# Autodesk Inventor assembly: Ствол
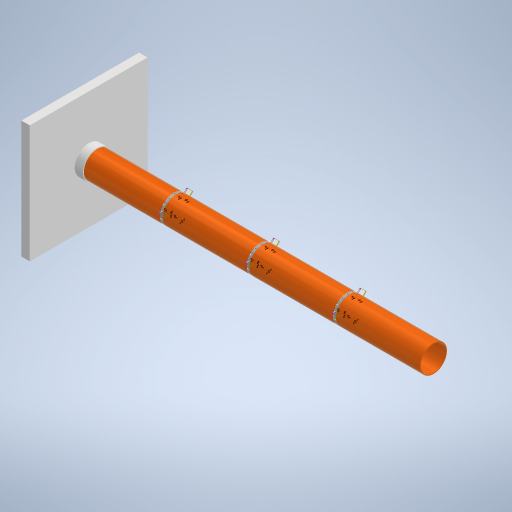
[picture p0: Inventor's stored thumbnail of the model, 512x512]
Saved by Autodesk Inventor 2023 (Build 270158000, 158)
## iProperties
Created: 2024-01-16
Part Number: Ствол
Document SubType Name: Assembly
Designer: liza
Author: liza
## Documents named in this file (6)
- C:\Fox_Crow\Work\Crow_Sborka\Ствол.iam
- C:\Fox_Crow\Work\Crow_Sborka\труба.ipt
- C:\Fox_Crow\Work\Crow_Sborka\внутренний соеденитель труб2.ipt
- C:\Fox_Crow\Work\Crow_Sborka\ветка.ipt
- C:\Fox_Crow\Work\Crow_Sborka\крепеж крышки+доска.ipt
- C:\Fox_Crow\Work\Crow_Sborka\трубка ветка.ipt
## Components (24 placed, 5 different names)
1. ветка:1 — Заподлицо:2
2. крепеж крышки+доска:1 — Цилиндрический:1, С поворотом:1
3. труба:5 — С поворотом:2
4. труба:2 — Совмещение:1, Совмещение:2, Заподлицо:1, Совмещение:3, Совмещение:4, Цилиндрический:1, С поворотом:1
5. труба:3
6. труба:4 — С поворотом:2
7. внутренний соеденитель труб2:1 — Совмещение:3, Совмещение:4, Цилиндрический:2, Цилиндрический:3
8. трубка ветка:1 — Цилиндрический:2, Цилиндрический:3
9. внутренний соеденитель труб2:2
10. трубка ветка:3
11. внутренний соеденитель труб2:3
12. трубка ветка:4
13. внутренний соеденитель труб2:4
14. трубка ветка:5
15. внутренний соеденитель труб2:5
16. трубка ветка:6
17. внутренний соеденитель труб2:6
18. трубка ветка:7
19. внутренний соеденитель труб2:7
20. трубка ветка:8
21. внутренний соеденитель труб2:8
22. трубка ветка:9
23. внутренний соеденитель труб2:9
24. трубка ветка:10
## Component patterns: (3 elements, first: труба:2), (1 elements), МассивКомп 2:2 (1 elements), МассивКомп 2:3 (1 elements), (3 elements, first: внутренний соеденитель труб2:1 + трубка ветка:1), МассивКомп 1:2 (3 elements), МассивКомп 1:3 (3 elements)
## Relationships (11: Mate 4, CylindricalJoint 3, Flush 2, RevoluteJoint 2)
- Совмещение:1 [Mate]: труба:2
- Совмещение:2 [Mate]: труба:2
- Заподлицо:1 [Flush]: труба:2
- Совмещение:3 [Mate]: труба:2 ↔ внутренний соеденитель труб2:1
- Совмещение:4 [Mate]: труба:2 ↔ внутренний соеденитель труб2:1
- Заподлицо:2 [Flush]: ветка:1
- Цилиндрический:1 [CylindricalJoint]: крепеж крышки+доска:1 ↔ труба:2
- С поворотом:1 [RevoluteJoint]: крепеж крышки+доска:1 ↔ труба:2
- С поворотом:2 [RevoluteJoint] (15 mm): труба:5 ↔ труба:4
- Цилиндрический:2 [CylindricalJoint]: внутренний соеденитель труб2:1 ↔ трубка ветка:1
- Цилиндрический:3 [CylindricalJoint]: внутренний соеденитель труб2:1 ↔ трубка ветка:1
